# Autodesk Inventor assembly: ForceMeterAsmy
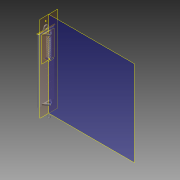
[picture p0: Inventor's stored thumbnail of the model, 180x180]
Saved by Autodesk Inventor 2012 SP2 (Build 160219200, 219)
## iProperties
Created: 2014-02-08
Part Number: ForceMeterAsmy
Document SubType Name: Assembly
Designer: 1
Author: 1
## Documents named in this file (4)
- D:\p3_metod1580library\figures\sources\M7-BallRotatorMachine\ForceMeterAsmy.iam
- D:\p3_metod1580library\figures\sources\M7-BallRotatorMachine\ForceMeterCasing.ipt
- D:\p3_metod1580library\figures\sources\M7-BallRotatorMachine\ForceMeterSpring.ipt
- D:\p3_metod1580library\figures\sources\M7-BallRotatorMachine\Ball.ipt
## Components (3 placed, 3 different names)
1. ForceMeterCasing:1 — Mate:1, Angle:1, Flush:3, Flush:4
2. ForceMeterSpring:1 — Flush:1, Flush:2, Flush:3, Flush:4
3. Ball:1 — Flush:5
## Relationships (10: Flush 5, Mate 3, Angle 2)
- Mate:1: ForceMeterCasing:1
- Mate:2
- Angle:1 (0 deg): ForceMeterCasing:1
- Mate:3
- Angle:2 (90 deg)
- Flush:1: ForceMeterSpring:1
- Flush:2: ForceMeterSpring:1
- Flush:3: ForceMeterCasing:1 ↔ ForceMeterSpring:1
- Flush:4: ForceMeterCasing:1 ↔ ForceMeterSpring:1
- Flush:5: Ball:1
